# Autodesk Inventor assembly: робот - сборка фулл
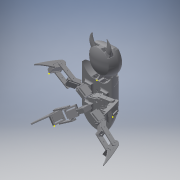
[picture p0: Inventor's stored thumbnail of the model, 180x180]
Saved by Autodesk Inventor 2019 (Build 230136000, 136)
## iProperties
Created: 2019-09-07
Part Number: робот - сборка фулл
Material: Типовые
Document SubType Name: Assembly
Designer: Iliga
Author: Iliga
## Documents named in this file (7)
- C:\Users\Iliga\Desktop\робот\робот - сборка фулл.iam
- C:\Users\Iliga\Desktop\робот\тело.ipt
- C:\Users\Iliga\Desktop\робот\двигатель.ipt
- C:\Users\Iliga\Desktop\робот\правое надкрылье.ipt
- C:\Users\Iliga\Desktop\робот\голова - сборка.iam
- C:\Users\Iliga\Desktop\робот\левая лапа - сборка.iam
- C:\Users\Iliga\Desktop\робот\правая лапа - сборка.iam
## Components (8 placed, 6 different names)
1. тело основа:1 — Совмещение:1, Совмещение:2, Совмещение:3, Заподлицо:1, Совмещение:5, Совмещение:8, Совмещение:10, Совмещение:11, Совмещение:12, Совмещение:13, Совмещение:14, Совмещение:15, Совмещение:16, Совмещение:17
2. двигатель:1 — Совмещение:1, Совмещение:2, Совмещение:3, Совмещение:6, Совмещение:7
3. правое надкрылье:1 — Заподлицо:1, Совмещение:5, Совмещение:17
4. голова - сборка:1 [sub-assembly] — Совмещение:6, Совмещение:7
5. лапа:1 [sub-assembly] — Совмещение:11, Совмещение:12
6. лапа:2 [sub-assembly] — Совмещение:8, Совмещение:10
7. правая лапа - сборка:1 [sub-assembly] — Совмещение:13, Совмещение:14
8. правая лапа - сборка:2 [sub-assembly] — Совмещение:15, Совмещение:16
## Relationships (16: Mate 15, Flush 1)
- Совмещение:1 [Mate]: тело основа:1 ↔ двигатель:1
- Совмещение:2 [Mate]: тело основа:1 ↔ двигатель:1
- Совмещение:3 [Mate]: тело основа:1 ↔ двигатель:1
- Заподлицо:1 [Flush]: тело основа:1 ↔ правое надкрылье:1
- Совмещение:5 [Mate]: тело основа:1 ↔ правое надкрылье:1
- Совмещение:6 [Mate]: двигатель:1 ↔ голова - сборка:1
- Совмещение:7 [Mate]: двигатель:1 ↔ голова - сборка:1
- Совмещение:8 [Mate]: тело основа:1 ↔ лапа:2
- Совмещение:10 [Mate]: тело основа:1 ↔ лапа:2
- Совмещение:11 [Mate]: тело основа:1 ↔ лапа:1
- Совмещение:12 [Mate]: тело основа:1 ↔ лапа:1
- Совмещение:13 [Mate]: тело основа:1 ↔ правая лапа - сборка:1
- Совмещение:14 [Mate]: тело основа:1 ↔ правая лапа - сборка:1
- Совмещение:15 [Mate]: тело основа:1 ↔ правая лапа - сборка:2
- Совмещение:16 [Mate]: тело основа:1 ↔ правая лапа - сборка:2
- Совмещение:17 [Mate]: тело основа:1 ↔ правое надкрылье:1
